# Autodesk Inventor assembly: motagem_base
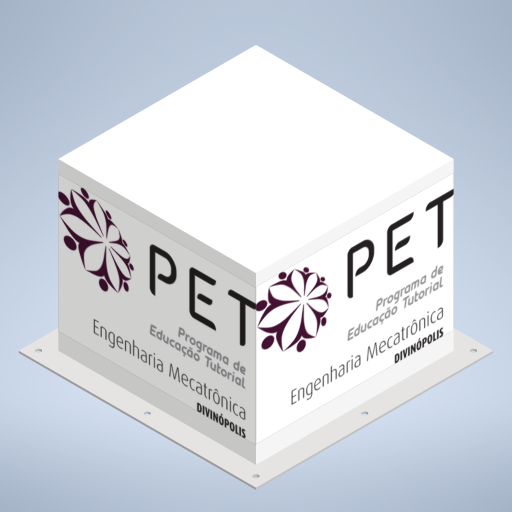
[picture p0: Inventor's stored thumbnail of the model, 512x512]
Saved by Autodesk Inventor 2023 (Build 270158000, 158)
## iProperties
Created: 2023-03-07
Part Number: motagem_base
Document SubType Name: Assembly
Designer: klebe
Author: klebe
## Documents named in this file (2)
- C:\Users\klebe\OneDrive\Documents\GitHub\Sala-braquiterapia\Sala de Braquiterapia\Inventor\Base Robos\motagem_base.iam
- C:\Users\klebe\OneDrive\Documents\GitHub\Sala-braquiterapia\Sala de Braquiterapia\Inventor\Base Robos\parte1.ipt
## Components (1 placed, 1 different names)
1. parte1:1 — Mate:1, Mate:2, Mate:3
## Relationships (3: Mate 3)
- Mate:1: parte1:1
- Mate:2: parte1:1
- Mate:3: parte1:1
